# Autodesk Inventor assembly: Assembly_final
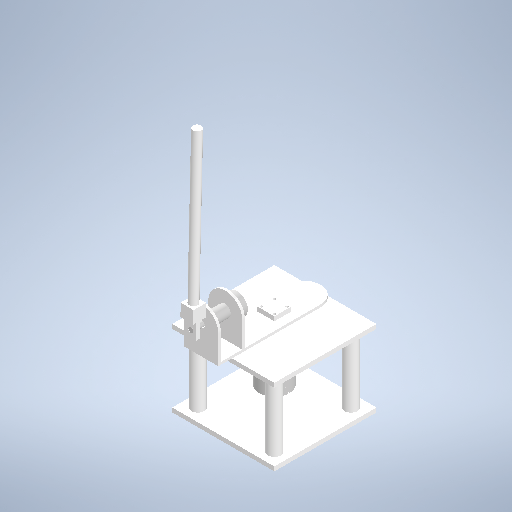
[picture p0: Inventor's stored thumbnail of the model, 512x512]
Saved by Autodesk Inventor 2025.3 (Build 293356000, 356)
## iProperties
Created: 2025-07-22
Part Number: Assembly_final
Document SubType Name: Assembly
Designer: KEVIN
Author: KEVIN
## Documents named in this file (8)
- C:\Users\KEVIN\OneDrive\Documentos\modern_control_project\inverted-pendulum\cad\Assembly_final.iam
- C:\Users\KEVIN\OneDrive\Documentos\modern_control_project\inverted-pendulum\cad\Base_engine.ipt
- C:\Users\KEVIN\OneDrive\Documentos\modern_control_project\inverted-pendulum\cad\Central_base.ipt
- C:\Users\KEVIN\OneDrive\Documentos\modern_control_project\inverted-pendulum\cad\pendulum.ipt
- C:\Users\KEVIN\OneDrive\Documentos\modern_control_project\inverted-pendulum\cad\DC_Motor_GA37RG_12V.ipt
- C:\Users\KEVIN\OneDrive\Documentos\modern_control_project\inverted-pendulum\cad\engine_coupling.ipt
- C:\Users\KEVIN\OneDrive\Documentos\modern_control_project\inverted-pendulum\cad\DC_motor_size_25.ipt
- C:\Users\KEVIN\OneDrive\Documentos\modern_control_project\inverted-pendulum\cad\pendulum_coupling.ipt
## Components (7 placed, 7 different names)
1. Base_engine:1 — Coincidencia:1, Coincidencia:2, Coincidencia:7, Coincidencia:8, Coincidencia:9, Coincidencia:10, Coincidencia:11, Coincidencia:12, Coincidencia:13, Coincidencia:16
2. Central_base:1 — Coincidencia:2, Coincidencia:3, Coincidencia:4
3. pendulum:1 — Coincidencia:1, Coincidencia:17, Nivelación:1
4. DC_Motor_GA37RG_12V:1 — Coincidencia:3, Coincidencia:4, Coincidencia:5, Coincidencia:6
5. engine_coupling:1 — Coincidencia:5, Coincidencia:6, Coincidencia:7, Coincidencia:8, Coincidencia:9, Coincidencia:10, Coincidencia:11
6. DC_motor_size_25:1 — Coincidencia:12, Coincidencia:13, Coincidencia:14, Coincidencia:15
7. pendulum_coupling:1 — Coincidencia:14, Coincidencia:15, Coincidencia:16, Coincidencia:17, Nivelación:1
## Relationships (18: Mate 17, Flush 1)
- Coincidencia:1 [Mate]: Base_engine:1 ↔ pendulum:1
- Coincidencia:2 [Mate]: Base_engine:1 ↔ Central_base:1
- Coincidencia:3 [Mate]: Central_base:1 ↔ DC_Motor_GA37RG_12V:1
- Coincidencia:4 [Mate]: Central_base:1 ↔ DC_Motor_GA37RG_12V:1
- Coincidencia:5 [Mate]: DC_Motor_GA37RG_12V:1 ↔ engine_coupling:1
- Coincidencia:6 [Mate]: DC_Motor_GA37RG_12V:1 ↔ engine_coupling:1
- Coincidencia:7 [Mate]: Base_engine:1 ↔ engine_coupling:1
- Coincidencia:8 [Mate]: Base_engine:1 ↔ engine_coupling:1
- Coincidencia:9 [Mate]: Base_engine:1 ↔ engine_coupling:1
- Coincidencia:10 [Mate]: Base_engine:1 ↔ engine_coupling:1
- Coincidencia:11 [Mate]: Base_engine:1 ↔ engine_coupling:1
- Coincidencia:12 [Mate]: Base_engine:1 ↔ DC_motor_size_25:1
- Coincidencia:13 [Mate]: Base_engine:1 ↔ DC_motor_size_25:1
- Coincidencia:14 [Mate]: DC_motor_size_25:1 ↔ pendulum_coupling:1
- Coincidencia:15 [Mate]: DC_motor_size_25:1 ↔ pendulum_coupling:1
- Coincidencia:16 [Mate]: Base_engine:1 ↔ pendulum_coupling:1
- Coincidencia:17 [Mate]: pendulum:1 ↔ pendulum_coupling:1
- Nivelación:1 [Flush]: pendulum:1 ↔ pendulum_coupling:1
